# Autodesk Inventor assembly: Additional_Building
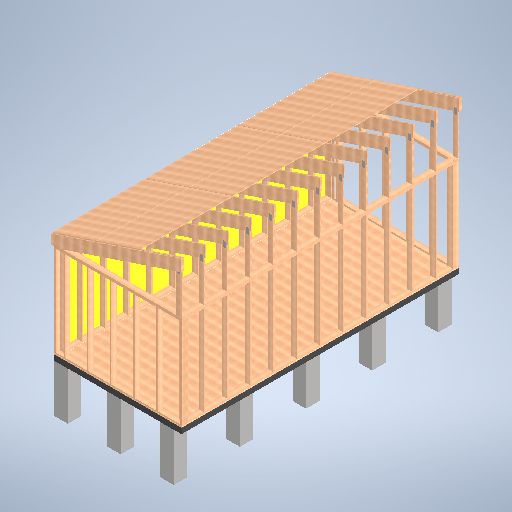
[picture p0: Inventor's stored thumbnail of the model, 512x512]
Saved by Autodesk Inventor 2025 (Build 290162010, 162A)
## iProperties
Created: 2024-08-02
Part Number: Additional_Building
Document SubType Name: Assembly
Designer: Tom
Author: Tom
## Documents named in this file (15)
- C:\Users\Tom\Documents\Inventor\Mobility\Additional_Building\Additional_Building.iam
- C:\Users\Tom\Documents\Inventor\Mobility\Additional_Building\Grid_Of_Piers.iam
- C:\Users\Tom\Documents\Inventor\Mobility\Additional_Building\Floor_System.iam
- C:\Users\Tom\Documents\Inventor\Mobility\Additional_Building\Walls.iam
- C:\Users\Tom\Documents\Inventor\Mobility\Additional_Building\Truss.iam
- C:\Users\Tom\Documents\Inventor\Mobility\Additional_Building\Sheathing_With_Dimensions_48_x_96_Inches.ipt
- C:\Users\Tom\Documents\Inventor\Mobility\Additional_Building\Sheathing_With_Dimensions_48_x_48_Inches.ipt
- C:\Users\Tom\Documents\Inventor\Mobility\Additional_Building\Sheathing_With_Dimensions_8.719_x_96_Inches.ipt
- C:\Users\Tom\Documents\Inventor\Mobility\Additional_Building\Siding.iam
- C:\Users\Tom\Documents\Inventor\Mobility\Additional_Building\Ender_Strip.ipt
- C:\Users\Tom\Documents\Inventor\Mobility\Additional_Building\OSB.ipt
- C:\Users\Tom\Documents\Inventor\Mobility\Additional_Building\Block_With_Width_21.75_Inches.ipt
- C:\Users\Tom\Documents\Inventor\Mobility\Additional_Building\Block_With_Width_22.5_Inches.ipt
- C:\Users\Tom\Documents\Inventor\Mobility\Additional_Building\Fascia.ipt
- C:\Users\Tom\Documents\Inventor\Mobility\Additional_Building\Rafter.ipt
## Components (49 placed, 14 different names)
1. Grid_Of_Piers:1 [sub-assembly] — Mate:12, Mate:13, Flush:7
2. Floor_System:1 [sub-assembly] — Mate:12, Mate:13, Flush:7, Mate:14, Flush:8, Flush:9, Flush:14
3. Walls:1 [sub-assembly] — Mate:14, Flush:8, Flush:9, Flush:10, Mate:15, Flush:11, Flush:12, Mate:16, Flush:13, Mate:17, Flush:15, Mate:18, Flush:16, Mate:20, Mate:22, Mate:24, Flush:19, Flush:30
4. Sheathing_With_Dimensions_48_x_48_Inches:1 — Mate:18, Mate:19, Flush:16, Mate:21, Flush:17, Mate:25
5. Sheathing_With_Dimensions_48_x_48_Inches:2 — Mate:22, Mate:23, Flush:18
6. Siding:1 [sub-assembly] — Mate:26, Flush:20, Flush:21, Flush:22
7. Ender_Strip:1 — Mate:27, Mate:28, Flush:22
8. Fascia:1 — Mate:32, Flush:29, Flush:30
9. Rafter:1 — Mate:35, Flush:32, Flush:33
10. Rafter:2 — Mate:36, Flush:34, Flush:35
11. Truss:1 [sub-assembly] — Flush:10, Mate:15, Flush:11, Mate:36, Flush:34, Flush:35
12. Truss:2 [sub-assembly] — Mate:29, Flush:23, Flush:24, Flush:25, Flush:26, Mate:30, Mate:35, Flush:32, Flush:33
13. Truss:3 [sub-assembly] — Flush:12, Mate:16, Flush:13, Mate:31, Flush:27
14. Truss:4 [sub-assembly] — Flush:28
15. Truss:5 [sub-assembly]
16. Truss:6 [sub-assembly]
17. Truss:7 [sub-assembly]
18. Truss:8 [sub-assembly] — Mate:28
19. Truss:9 [sub-assembly]
20. Truss:10 [sub-assembly]
21. Truss:11 [sub-assembly]
22. Truss:12 [sub-assembly]
23. Truss:13 [sub-assembly]
24. Sheathing_With_Dimensions_48_x_96_Inches:1 — Mate:17, Flush:14, Flush:15, Mate:19, Mate:26, Flush:21
25. Sheathing_With_Dimensions_48_x_96_Inches:2 — Flush:20
26. Sheathing_With_Dimensions_48_x_96_Inches:3
27. Sheathing_With_Dimensions_48_x_96_Inches:4 — Mate:20, Mate:21, Flush:17
28. Sheathing_With_Dimensions_48_x_96_Inches:5 — Mate:23, Flush:18
29. Sheathing_With_Dimensions_8.719_x_96_Inches:1 — Mate:24, Mate:25, Flush:19
30. Sheathing_With_Dimensions_8.719_x_96_Inches:2 — Mate:27
31. Sheathing_With_Dimensions_8.719_x_96_Inches:3
32. OSB:1 — Mate:29, Flush:23, Flush:24
33. OSB:2
34. OSB:3
35. OSB:4
36. OSB:5
37. OSB:6
38. Block_With_Width_22.5_Inches:1 — Mate:31, Flush:27, Flush:28
39. Block_With_Width_22.5_Inches:2 — Flush:29
40. Block_With_Width_22.5_Inches:3
41. Block_With_Width_22.5_Inches:4
42. Block_With_Width_22.5_Inches:5
43. Block_With_Width_22.5_Inches:6
44. Block_With_Width_22.5_Inches:7
45. Block_With_Width_22.5_Inches:8
46. Block_With_Width_22.5_Inches:9
47. Block_With_Width_22.5_Inches:10
48. Block_With_Width_21.75_Inches:1 — Flush:25, Flush:26, Mate:30, Mate:32
49. Block_With_Width_21.75_Inches:2
## Component patterns: (2 elements, first: Truss:1), (11 elements, first: Truss:3), (3 elements, first: Sheathing_With_Dimensions_48_x_96_Inches:1), (2 elements, first: Sheathing_With_Dimensions_48_x_96_Inches:4), (3 elements, first: Sheathing_With_Dimensions_8.719_x_96_Inches:1), (6 elements, first: OSB:1), (10 elements, first: Block_With_Width_22.5_Inches:1), (2 elements, first: Block_With_Width_21.75_Inches:1)
## Relationships (51: Flush 28, Mate 23)
- Mate:12: Grid_Of_Piers:1 ↔ Floor_System:1
- Mate:13: Grid_Of_Piers:1 ↔ Floor_System:1
- Flush:7: Grid_Of_Piers:1 ↔ Floor_System:1
- Mate:14: Floor_System:1 ↔ Walls:1
- Flush:8: Floor_System:1 ↔ Walls:1
- Flush:9: Floor_System:1 ↔ Walls:1
- Flush:10: Walls:1 ↔ Truss:1
- Mate:15: Walls:1 ↔ Truss:1
- Flush:11: Walls:1 ↔ Truss:1
- Flush:12: Walls:1 ↔ Truss:3
- Mate:16: Walls:1 ↔ Truss:3
- Flush:13 (590.55 mm): Walls:1 ↔ Truss:3
- Mate:17: Walls:1 ↔ Sheathing_With_Dimensions_48_x_96_Inches:1
- Flush:14 (-15.875 mm): Floor_System:1 ↔ Sheathing_With_Dimensions_48_x_96_Inches:1
- Flush:15: Walls:1 ↔ Sheathing_With_Dimensions_48_x_96_Inches:1
- Mate:18: Walls:1 ↔ Sheathing_With_Dimensions_48_x_48_Inches:1
- Mate:19: Sheathing_With_Dimensions_48_x_48_Inches:1 ↔ Sheathing_With_Dimensions_48_x_96_Inches:1
- Flush:16: Walls:1 ↔ Sheathing_With_Dimensions_48_x_48_Inches:1
- Mate:20: Walls:1 ↔ Sheathing_With_Dimensions_48_x_96_Inches:4
- Mate:21: Sheathing_With_Dimensions_48_x_48_Inches:1 ↔ Sheathing_With_Dimensions_48_x_96_Inches:4
- Flush:17: Sheathing_With_Dimensions_48_x_48_Inches:1 ↔ Sheathing_With_Dimensions_48_x_96_Inches:4
- Mate:22: Walls:1 ↔ Sheathing_With_Dimensions_48_x_48_Inches:2
- Mate:23: Sheathing_With_Dimensions_48_x_48_Inches:2 ↔ Sheathing_With_Dimensions_48_x_96_Inches:5
- Flush:18: Sheathing_With_Dimensions_48_x_48_Inches:2 ↔ Sheathing_With_Dimensions_48_x_96_Inches:5
- Mate:24: Walls:1 ↔ Sheathing_With_Dimensions_8.719_x_96_Inches:1
- Mate:25: Sheathing_With_Dimensions_48_x_48_Inches:1 ↔ Sheathing_With_Dimensions_8.719_x_96_Inches:1
- Flush:19: Walls:1 ↔ Sheathing_With_Dimensions_8.719_x_96_Inches:1
- Mate:26: Siding:1 ↔ Sheathing_With_Dimensions_48_x_96_Inches:1
- Flush:20 (-6.35 mm): Siding:1 ↔ Sheathing_With_Dimensions_48_x_96_Inches:2
- Flush:21 (-15.875 mm): Siding:1 ↔ Sheathing_With_Dimensions_48_x_96_Inches:1
- Mate:27: Ender_Strip:1 ↔ Sheathing_With_Dimensions_8.719_x_96_Inches:2
- Mate:28: Ender_Strip:1 ↔ Truss:8
- Flush:22: Siding:1 ↔ Ender_Strip:1
- Mate:29: Truss:2 ↔ OSB:1
- Flush:23: Truss:2 ↔ OSB:1
- Flush:24: Truss:2 ↔ OSB:1
- Flush:25: Truss:2 ↔ Block_With_Width_21.75_Inches:1
- Flush:26: Truss:2 ↔ Block_With_Width_21.75_Inches:1
- Mate:30: Truss:2 ↔ Block_With_Width_21.75_Inches:1
- Mate:31: Truss:3 ↔ Block_With_Width_22.5_Inches:1
- Flush:27: Truss:3 ↔ Block_With_Width_22.5_Inches:1
- Flush:28: Truss:4 ↔ Block_With_Width_22.5_Inches:1
- Mate:32: Fascia:1 ↔ Block_With_Width_21.75_Inches:1
- Flush:29 (-6.35 mm): Fascia:1 ↔ Block_With_Width_22.5_Inches:2
- Flush:30: Walls:1 ↔ Fascia:1
- Mate:35: Rafter:1 ↔ Truss:2
- Flush:32: Rafter:1 ↔ Truss:2
- Flush:33: Rafter:1 ↔ Truss:2
- Mate:36: Rafter:2 ↔ Truss:1
- Flush:34: Rafter:2 ↔ Truss:1
- Flush:35: Rafter:2 ↔ Truss:1
